# Autodesk Inventor assembly: body_frame
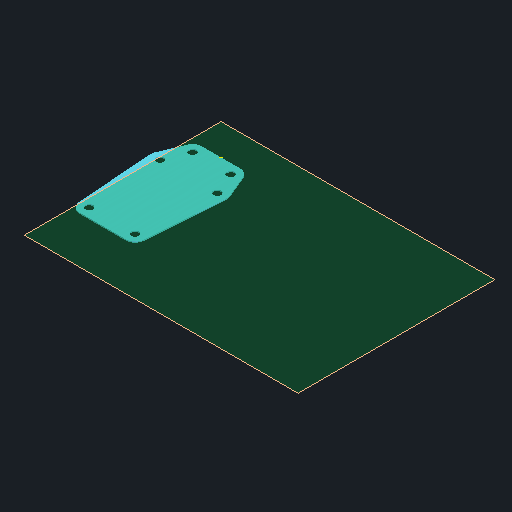
[picture p0: Inventor's stored thumbnail of the model, 512x512]
Saved by Autodesk Inventor 2026 (Build 300175000, 175)
## iProperties
Created: 2026-04-26
Part Number: body_frame
Document SubType Name: Assembly
Designer: user
Mass: 1256.55 g
Surface Area: 1105.69 cm^2
Volume: 160.07 cm^3
Author: user
## Documents named in this file (2)
- C:\Users\user\Documents\spider_metal\body_frame.iam
- C:\Users\user\Documents\spider_metal\body_parts\body_composition.ipt
## Components (1 placed, 1 different names)
1. body_composition:1 — Совмещение:2, Заподлицо:1, Совмещение:3
## Relationships (3: Mate 2, Flush 1)
- Совмещение:2 [Mate]: body_composition:1
- Заподлицо:1 [Flush]: body_composition:1
- Совмещение:3 [Mate]: body_composition:1
